# Autodesk Inventor assembly: Kitchen 2
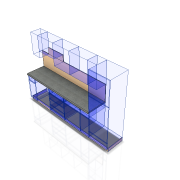
[picture p0: Inventor's stored thumbnail of the model, 180x180]
Saved by Autodesk Inventor 2024 (Build 280153000, 153)
## iProperties
Created: 2017-05-02
Part Number: Kitchen 2
Document SubType Name: Assembly
Designer: SauliusD
Author: SauliusD
## Documents named in this file (8)
- C:\W4INV 2024 Design\PROJECTS\Samples\Kitchen design\Kitchen.iam
- C:\W4INV 2024 Design\PROJECTS\Samples\Kitchen design\Flat.ipt
- C:\W4INV 2024 Design\PROJECTS\Samples\Kitchen design\Big Wall Panel.ipt
- C:\W4INV 2024 Design\PROJECTS\Samples\Kitchen design\Small Wall Panel.ipt
- C:\W4INV 2024 Design\PROJECTS\Samples\Kitchen design\Plynth Panel1.ipt
- C:\W4INV 2024 Design\PROJECTS\Samples\Kitchen design\Plynth Panel2.ipt
- C:\W4INV 2024 Design\PROJECTS\Samples\Kitchen design\Plynth Panel3.ipt
- C:\W4INV 2024 Design\PROJECTS\Samples\Kitchen design\Desktop.ipt
## Components (7 placed, 7 different names)
1. Flat:1 — Flush:1, Flush:2, Flush:3
2. Big Wall Panel:1
3. Small Wall Panel:1
4. Plynth Panel1:1
5. Plynth Panel2:1
6. Plynth Panel3:1
7. Desktop:1
## Relationships (3: Flush 3)
- Flush:1: Flat:1
- Flush:2: Flat:1
- Flush:3: Flat:1
